# Autodesk Inventor assembly: Adafruit MPRLS Ported Pressure Sensor Breakout with pins
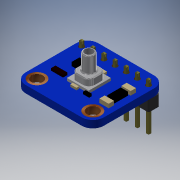
[picture p0: Inventor's stored thumbnail of the model, 180x180]
Saved by Autodesk Inventor 2019.3 (Build 233278000, 278)
## iProperties
Created: 2020-04-23
Part Number: Adafruit MPRLS Ported Pressure Sensor Breakout with pins
Document SubType Name: Assembly
Designer: rjpc1
Author: rjpc1
## Documents named in this file (3)
- C:\Users\rjpc1\Documents\Universidad del valle\Proyectos\Respirador\Adafruit MPRLS Ported Pressure Sensor Breakout with pins.iam
- C:\Users\rjpc1\Documents\Universidad del valle\Proyectos\Respirador\Adafruit MPRLS Ported Pressure Sensor Breakout.ipt
- C:\Users\rjpc1\Documents\Universidad del valle\Proyectos\Respirador\Male Header.ipt
## Components (8 placed, 2 different names)
1. Adafruit MPRLS Ported Pressure Sensor Breakout:1 — Mate:1, Flush:1, Flush:2, Mate:2, Mate:3, Mate:4, Mate:5, Mate:6, Mate:7
2. Male Header:1 — Mate:7, Mate:9, Mate:10, Flush:4, Flush:5
3. Male Header:2 — Mate:6, Mate:11, Mate:12, Flush:6, Flush:7
4. Male Header:3 — Mate:5, Mate:13, Flush:8
5. Male Header:4 — Mate:4, Mate:12, Mate:13, Flush:7, Flush:8
6. Male Header:5 — Mate:3, Mate:10, Mate:11, Flush:5, Flush:6
7. Male Header:6 — Mate:2, Mate:8, Mate:9, Flush:3, Flush:4
8. Male Header:7 — Mate:1, Flush:1, Flush:2, Mate:8, Flush:3
## Relationships (21: Mate 13, Flush 8)
- Mate:1: Adafruit MPRLS Ported Pressure Sensor Breakout:1 ↔ Male Header:7
- Flush:1: Adafruit MPRLS Ported Pressure Sensor Breakout:1 ↔ Male Header:7
- Flush:2 (1.25 mm): Adafruit MPRLS Ported Pressure Sensor Breakout:1 ↔ Male Header:7
- Mate:2: Adafruit MPRLS Ported Pressure Sensor Breakout:1 ↔ Male Header:6
- Mate:3: Adafruit MPRLS Ported Pressure Sensor Breakout:1 ↔ Male Header:5
- Mate:4: Adafruit MPRLS Ported Pressure Sensor Breakout:1 ↔ Male Header:4
- Mate:5: Adafruit MPRLS Ported Pressure Sensor Breakout:1 ↔ Male Header:3
- Mate:6: Adafruit MPRLS Ported Pressure Sensor Breakout:1 ↔ Male Header:2
- Mate:7: Adafruit MPRLS Ported Pressure Sensor Breakout:1 ↔ Male Header:1
- Mate:8: Male Header:6 ↔ Male Header:7
- Mate:9: Male Header:1 ↔ Male Header:6
- Mate:10: Male Header:1 ↔ Male Header:5
- Mate:11: Male Header:2 ↔ Male Header:5
- Mate:12: Male Header:2 ↔ Male Header:4
- Mate:13: Male Header:3 ↔ Male Header:4
- Flush:3: Male Header:6 ↔ Male Header:7
- Flush:4: Male Header:1 ↔ Male Header:6
- Flush:5: Male Header:1 ↔ Male Header:5
- Flush:6: Male Header:2 ↔ Male Header:5
- Flush:7: Male Header:2 ↔ Male Header:4
- Flush:8: Male Header:3 ↔ Male Header:4
